# Autodesk Inventor assembly: centre wing
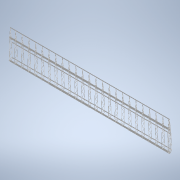
[picture p0: Inventor's stored thumbnail of the model, 180x180]
Saved by Autodesk Inventor 2022 (Build 260153000, 153)
## iProperties
Created: 2021-03-09
Part Number: centre wing
Document SubType Name: Assembly
Designer: Ferdinand Hubbard
Author: Ferdinand Hubbard
## Documents named in this file (6)
- C:\Users\Ferdinand Hubbard\Desktop\solarplane\cad\centre wing section.iam
- C:\Users\Ferdinand Hubbard\Desktop\solarplane\cad\tubes\normal tubes\18mm tube.ipt
- C:\Users\Ferdinand Hubbard\Desktop\solarplane\cad\tubes\normal tubes\15mm tube.ipt
- C:\Users\Ferdinand Hubbard\Desktop\solarplane\cad\airfoils\full airfoil\full airfoil blueprint 19 mm.ipt
- C:\Users\Ferdinand Hubbard\Desktop\solarplane\cad\airfoils\full airfoil\full airfoil blueprint 16 mm.ipt
- C:\Users\Ferdinand Hubbard\Desktop\solarplane\cad\wood 5 5 1952.ipt
## Components (37 placed, 5 different names)
1. 18mm tube:2 — Mate:1, Mate:2, Mate:5, Mate:6
2. 15mm tube:2 — Mate:1, Mate:2, Mate:82, Flush:4
3. 18mm tube:3 — Flush:2, Angle:1, Mate:98
4. 15mm tube:3 — Mate:5, Mate:6, Mate:98
5. 18mm tube:4
6. 15mm tube:4 — Mate:81, Flush:3
7. 18mm tube:5 — Mate:23, Flush:1, Angle:2, Mate:99, Flush:11
8. 15mm tube:5 — Mate:99
9. wood 5 5 1952:1 — Mate:90, Mate:91, Flush:7, Mate:96, Mate:97, Flush:10
10. wood 5 5 1952:2 — Mate:86, Mate:87, Flush:5, Mate:92, Mate:93, Flush:8
11. wood 5 5 1952:3 — Mate:88, Mate:89, Flush:6, Mate:94, Mate:95, Flush:9
12. full airfoil blueprint 19 mm:1 — Mate:13, Mate:14, Mate:15, Mate:23, Flush:1, Flush:2, Mate:86, Mate:87, Flush:5, Mate:88, Mate:89, Flush:6, Mate:90, Mate:91, Flush:7, Angle:1, Mate:100, Mate:101
13. full airfoil blueprint 19 mm:2 — Mate:13, Mate:14, Mate:15, Mate:19, Mate:20, Mate:21, Angle:2
14. full airfoil blueprint 19 mm:3 — Mate:19, Mate:20, Mate:21
15. full airfoil blueprint 19 mm:4 — Mate:30, Mate:31, Mate:32
16. full airfoil blueprint 19 mm:5 — Mate:30, Mate:31, Mate:32
17. full airfoil blueprint 19 mm:6
18. full airfoil blueprint 19 mm:7 — Mate:42, Mate:43, Mate:44
19. full airfoil blueprint 16 mm:1 — Mate:33, Mate:34, Mate:35, Mate:42, Mate:43, Mate:44
20. full airfoil blueprint 16 mm:2 — Mate:33, Mate:34, Mate:35, Mate:39, Mate:40, Mate:41
21. full airfoil blueprint 16 mm:3 — Mate:39, Mate:40, Mate:41
22. full airfoil blueprint 16 mm:4 — Mate:45, Mate:46, Mate:47
23. full airfoil blueprint 16 mm:5 — Mate:45, Mate:46, Mate:47, Mate:63, Mate:64, Mate:65
24. full airfoil blueprint 19 mm:8 — Mate:63, Mate:64, Mate:65
25. full airfoil blueprint 19 mm:9
26. full airfoil blueprint 19 mm:10
27. full airfoil blueprint 19 mm:11
28. full airfoil blueprint 19 mm:12
29. full airfoil blueprint 19 mm:13 — Mate:78, Mate:79, Mate:80
30. full airfoil blueprint 16 mm:6 — Mate:78, Mate:79, Mate:80
31. full airfoil blueprint 16 mm:7
32. full airfoil blueprint 16 mm:8
33. full airfoil blueprint 16 mm:9
34. full airfoil blueprint 16 mm:10 — Mate:83, Mate:84, Mate:85
35. full airfoil blueprint 16 mm:11 — Mate:81, Mate:82, Flush:3, Flush:4, Mate:92, Mate:93, Flush:8, Mate:94, Mate:95, Flush:9, Mate:96, Mate:97, Flush:10
36. full airfoil blueprint 16 mm:12 — Mate:83, Mate:84, Mate:85
37. full airfoil blueprint 19 mm:14 — Flush:11, Mate:100, Mate:101
## Relationships (111: Mate 98, Flush 11, Angle 2)
- Mate:1: 18mm tube:2 ↔ 15mm tube:2
- Mate:2: 18mm tube:2 ↔ 15mm tube:2
- [Mate]: 18mm tube:3 ↔ 15mm tube:3
- Mate:5: 18mm tube:2 ↔ 15mm tube:3
- Mate:6: 18mm tube:2 ↔ 15mm tube:3
- [Mate]: 18mm tube:4 ↔ 15mm tube:4
- [Mate]: 18mm tube:4 ↔ 15mm tube:4
- [Mate]: 18mm tube:5 ↔ 15mm tube:5
- [Mate]: 18mm tube:4 ↔ 15mm tube:5
- [Mate]: 18mm tube:4 ↔ 15mm tube:5
- Mate:13 (80 mm): full airfoil blueprint 19 mm:1 ↔ full airfoil blueprint 19 mm:2
- Mate:14: full airfoil blueprint 19 mm:1 ↔ full airfoil blueprint 19 mm:2
- Mate:15: full airfoil blueprint 19 mm:1 ↔ full airfoil blueprint 19 mm:2
- [Mate] (80 mm): full airfoil blueprint 19 mm:3 ↔ full airfoil blueprint 19 mm:4
- [Mate]: full airfoil blueprint 19 mm:3 ↔ full airfoil blueprint 19 mm:4
- [Mate]: full airfoil blueprint 19 mm:3 ↔ full airfoil blueprint 19 mm:4
- Mate:19 (80 mm): full airfoil blueprint 19 mm:2 ↔ full airfoil blueprint 19 mm:3
- Mate:20: full airfoil blueprint 19 mm:2 ↔ full airfoil blueprint 19 mm:3
- Mate:21: full airfoil blueprint 19 mm:2 ↔ full airfoil blueprint 19 mm:3
- Mate:23: 18mm tube:5 ↔ full airfoil blueprint 19 mm:1
- Flush:1: 18mm tube:5 ↔ full airfoil blueprint 19 mm:1
- Flush:2: 18mm tube:3 ↔ full airfoil blueprint 19 mm:1
- [Mate] (80 mm): full airfoil blueprint 19 mm:6 ↔ full airfoil blueprint 19 mm:7
- [Mate]: full airfoil blueprint 19 mm:6 ↔ full airfoil blueprint 19 mm:7
- [Mate]: full airfoil blueprint 19 mm:6 ↔ full airfoil blueprint 19 mm:7
- [Mate] (80 mm): full airfoil blueprint 19 mm:5 ↔ full airfoil blueprint 19 mm:6
- [Mate]: full airfoil blueprint 19 mm:5 ↔ full airfoil blueprint 19 mm:6
- [Mate]: full airfoil blueprint 19 mm:5 ↔ full airfoil blueprint 19 mm:6
- Mate:30 (80 mm): full airfoil blueprint 19 mm:4 ↔ full airfoil blueprint 19 mm:5
- Mate:31: full airfoil blueprint 19 mm:4 ↔ full airfoil blueprint 19 mm:5
- Mate:32: full airfoil blueprint 19 mm:4 ↔ full airfoil blueprint 19 mm:5
- Mate:33 (80 mm): full airfoil blueprint 16 mm:1 ↔ full airfoil blueprint 16 mm:2
- Mate:34: full airfoil blueprint 16 mm:1 ↔ full airfoil blueprint 16 mm:2
- Mate:35: full airfoil blueprint 16 mm:1 ↔ full airfoil blueprint 16 mm:2
- [Mate] (80 mm): full airfoil blueprint 16 mm:3 ↔ full airfoil blueprint 16 mm:4
- [Mate]: full airfoil blueprint 16 mm:3 ↔ full airfoil blueprint 16 mm:4
- [Mate]: full airfoil blueprint 16 mm:3 ↔ full airfoil blueprint 16 mm:4
- Mate:39 (80 mm): full airfoil blueprint 16 mm:2 ↔ full airfoil blueprint 16 mm:3
- Mate:40: full airfoil blueprint 16 mm:2 ↔ full airfoil blueprint 16 mm:3
- Mate:41: full airfoil blueprint 16 mm:2 ↔ full airfoil blueprint 16 mm:3
- Mate:42 (80 mm): full airfoil blueprint 19 mm:7 ↔ full airfoil blueprint 16 mm:1
- Mate:43: full airfoil blueprint 19 mm:7 ↔ full airfoil blueprint 16 mm:1
- Mate:44: full airfoil blueprint 19 mm:7 ↔ full airfoil blueprint 16 mm:1
- Mate:45 (80 mm): full airfoil blueprint 16 mm:4 ↔ full airfoil blueprint 16 mm:5
- Mate:46: full airfoil blueprint 16 mm:4 ↔ full airfoil blueprint 16 mm:5
- Mate:47: full airfoil blueprint 16 mm:4 ↔ full airfoil blueprint 16 mm:5
- [Mate] (80 mm): full airfoil blueprint 19 mm:9 ↔ full airfoil blueprint 19 mm:10
- [Mate]: full airfoil blueprint 19 mm:9 ↔ full airfoil blueprint 19 mm:10
- [Mate]: full airfoil blueprint 19 mm:9 ↔ full airfoil blueprint 19 mm:10
- [Mate] (80 mm): full airfoil blueprint 19 mm:8 ↔ full airfoil blueprint 19 mm:9
- [Mate]: full airfoil blueprint 19 mm:8 ↔ full airfoil blueprint 19 mm:9
- [Mate]: full airfoil blueprint 19 mm:8 ↔ full airfoil blueprint 19 mm:9
- [Mate] (80 mm): full airfoil blueprint 19 mm:12 ↔ full airfoil blueprint 19 mm:13
- [Mate]: full airfoil blueprint 19 mm:12 ↔ full airfoil blueprint 19 mm:13
- [Mate]: full airfoil blueprint 19 mm:12 ↔ full airfoil blueprint 19 mm:13
- [Mate] (80 mm): full airfoil blueprint 19 mm:11 ↔ full airfoil blueprint 19 mm:12
- [Mate]: full airfoil blueprint 19 mm:11 ↔ full airfoil blueprint 19 mm:12
- [Mate]: full airfoil blueprint 19 mm:11 ↔ full airfoil blueprint 19 mm:12
- [Mate] (80 mm): full airfoil blueprint 19 mm:10 ↔ full airfoil blueprint 19 mm:11
- [Mate]: full airfoil blueprint 19 mm:10 ↔ full airfoil blueprint 19 mm:11
- [Mate]: full airfoil blueprint 19 mm:10 ↔ full airfoil blueprint 19 mm:11
- Mate:63 (80 mm): full airfoil blueprint 16 mm:5 ↔ full airfoil blueprint 19 mm:8
- Mate:64: full airfoil blueprint 16 mm:5 ↔ full airfoil blueprint 19 mm:8
- Mate:65: full airfoil blueprint 16 mm:5 ↔ full airfoil blueprint 19 mm:8
- [Mate] (80 mm): full airfoil blueprint 16 mm:6 ↔ full airfoil blueprint 16 mm:7
- [Mate]: full airfoil blueprint 16 mm:6 ↔ full airfoil blueprint 16 mm:7
- [Mate]: full airfoil blueprint 16 mm:6 ↔ full airfoil blueprint 16 mm:7
- [Mate] (80 mm): full airfoil blueprint 16 mm:8 ↔ full airfoil blueprint 16 mm:9
- [Mate]: full airfoil blueprint 16 mm:8 ↔ full airfoil blueprint 16 mm:9
- [Mate]: full airfoil blueprint 16 mm:8 ↔ full airfoil blueprint 16 mm:9
- [Mate] (80 mm): full airfoil blueprint 16 mm:7 ↔ full airfoil blueprint 16 mm:8
- [Mate]: full airfoil blueprint 16 mm:7 ↔ full airfoil blueprint 16 mm:8
- [Mate]: full airfoil blueprint 16 mm:7 ↔ full airfoil blueprint 16 mm:8
- [Mate] (80 mm): full airfoil blueprint 16 mm:9 ↔ full airfoil blueprint 16 mm:10
- [Mate]: full airfoil blueprint 16 mm:9 ↔ full airfoil blueprint 16 mm:10
- [Mate]: full airfoil blueprint 16 mm:9 ↔ full airfoil blueprint 16 mm:10
- Mate:78 (80 mm): full airfoil blueprint 19 mm:13 ↔ full airfoil blueprint 16 mm:6
- Mate:79: full airfoil blueprint 19 mm:13 ↔ full airfoil blueprint 16 mm:6
- Mate:80: full airfoil blueprint 19 mm:13 ↔ full airfoil blueprint 16 mm:6
- Mate:81: 15mm tube:4 ↔ full airfoil blueprint 16 mm:11
- Mate:82: 15mm tube:2 ↔ full airfoil blueprint 16 mm:11
- Flush:3 (12 mm): 15mm tube:4 ↔ full airfoil blueprint 16 mm:11
- Flush:4 (12 mm): 15mm tube:2 ↔ full airfoil blueprint 16 mm:11
- Mate:83 (80 mm): full airfoil blueprint 16 mm:10 ↔ full airfoil blueprint 16 mm:12
- Mate:84: full airfoil blueprint 16 mm:10 ↔ full airfoil blueprint 16 mm:12
- Mate:85: full airfoil blueprint 16 mm:10 ↔ full airfoil blueprint 16 mm:12
- Mate:86: wood 5 5 1952:2 ↔ full airfoil blueprint 19 mm:1
- Mate:87: wood 5 5 1952:2 ↔ full airfoil blueprint 19 mm:1
- Flush:5: wood 5 5 1952:2 ↔ full airfoil blueprint 19 mm:1
- Mate:88: wood 5 5 1952:3 ↔ full airfoil blueprint 19 mm:1
- Mate:89: wood 5 5 1952:3 ↔ full airfoil blueprint 19 mm:1
- Flush:6: wood 5 5 1952:3 ↔ full airfoil blueprint 19 mm:1
- Mate:90: wood 5 5 1952:1 ↔ full airfoil blueprint 19 mm:1
- Mate:91: wood 5 5 1952:1 ↔ full airfoil blueprint 19 mm:1
- Flush:7: wood 5 5 1952:1 ↔ full airfoil blueprint 19 mm:1
- Mate:92: wood 5 5 1952:2 ↔ full airfoil blueprint 16 mm:11
- Mate:93: wood 5 5 1952:2 ↔ full airfoil blueprint 16 mm:11
- Flush:8: wood 5 5 1952:2 ↔ full airfoil blueprint 16 mm:11
- Mate:94: wood 5 5 1952:3 ↔ full airfoil blueprint 16 mm:11
- Mate:95: wood 5 5 1952:3 ↔ full airfoil blueprint 16 mm:11
- Flush:9: wood 5 5 1952:3 ↔ full airfoil blueprint 16 mm:11
- Mate:96: wood 5 5 1952:1 ↔ full airfoil blueprint 16 mm:11
- Mate:97: wood 5 5 1952:1 ↔ full airfoil blueprint 16 mm:11
- Flush:10: wood 5 5 1952:1 ↔ full airfoil blueprint 16 mm:11
- Angle:1 (180 deg): 18mm tube:3 ↔ full airfoil blueprint 19 mm:1
- Mate:98: 18mm tube:3 ↔ 15mm tube:3
- Angle:2 (180 deg): 18mm tube:5 ↔ full airfoil blueprint 19 mm:2
- Mate:99: 18mm tube:5 ↔ 15mm tube:5
- Flush:11 (10 mm): 18mm tube:5 ↔ full airfoil blueprint 19 mm:14
- Mate:100: full airfoil blueprint 19 mm:1 ↔ full airfoil blueprint 19 mm:14
- Mate:101: full airfoil blueprint 19 mm:1 ↔ full airfoil blueprint 19 mm:14
## Named parameters: d100_d98 = 0 mm, d103_d97 = 0 mm, d104_d98 = 0 mm, d106_d100_d98 = 0 mm, d107_d101 = 0 mm, d108_d102 = 0 mm, d230_d227 = 80 mm, d231_d228 = 0 mm, d232_d229 = 0 mm, d240_d230_d227 = 80 mm, d241_d231_d228 = 0 mm, d242_d232_d229 = 0 mm, d243_d233 = 80 mm, d244_d234 = 0 mm, d245_d235 = 0 mm, d253_d250 = 80 mm, d254_d251 = 0 mm, d255_d252 = 0 mm, d268_d230_d227 = 80 mm, d269_d231_d228 = 0 mm, d270_d232_d229 = 0 mm, d271_d233 = 80 mm, d272_d234 = 0 mm, d273_d235 = 0 mm, d274_d240_d230_d227 = 80 mm, d275_d241_d231_d228 = 0 mm, d276_d242_d232_d229 = 0 mm, d277_d243_d233 = 80 mm, d278_d244_d234 = 0 mm, d279_d245_d235 = 0 mm, d280_d247 = 80 mm, d281_d248 = 0 mm, d282_d249 = 0 mm, d287_d250 = 80 mm, d288_d251 = 0 mm, d289_d252 = 0 mm, d290_d253_d250 = 80 mm, d291_d254_d251 = 0 mm, d292_d255_d252 = 0 mm, d293_d256 = 80 mm, d294_d257 = 0 mm, d295_d258 = 0 mm, d296_d265 = 80 mm, d297_d266 = 0 mm, d298_d267 = 0 mm
